# Autodesk Inventor assembly: L1 Gearbox Assembly
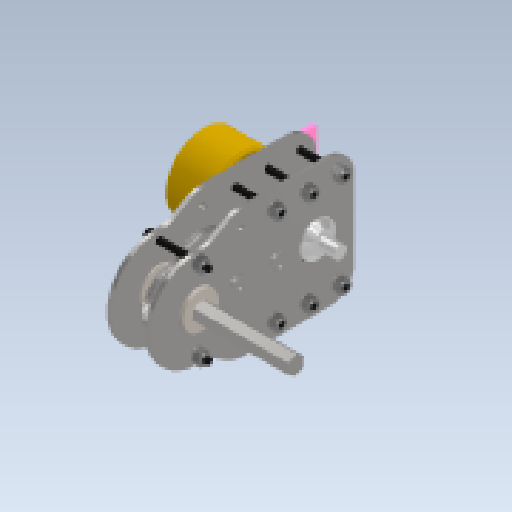
[picture p0: Inventor's stored thumbnail of the model, 512x512]
Saved by Autodesk Inventor 2023 (Build 270158000, 158)
## iProperties
Created: 2023-02-14
Part Number: L1 Gearbox Assembly
Document SubType Name: Assembly
Designer: Dave
Mass: 913.46 g
Surface Area: 1660.69 cm^2
Volume: 243.163 cm^3
Density: 3.75658 g/cm^3
Author: Dave
## Documents named in this file (16)
- C:\Users\Dave\Documents\GitHub\BehrendURCMechanical\CAD\Chassis V3\L1 Gearbox Assembly.iam
- C:\Users\Dave\Documents\GitHub\BehrendURCMechanical\CAD\Chassis\GearBox\Final Gears and Assemblies\CH-1-01-20T_Drive Gear.ipt
- C:\Users\Dave\Documents\GitHub\BehrendURCMechanical\CAD\Chassis\GearBox\Final Gears and Assemblies\CH-1-01-60T_Output.ipt
- C:\Users\Dave\Documents\GitHub\BehrendURCMechanical\CAD\Chassis\GearBox\Final Gears and Assemblies\CH-1-01-20T_Idler.ipt
- C:\Users\Dave\Documents\GitHub\BehrendURCMechanical\CAD\Chassis\GearBox\Final Gears and Assemblies\CH-1-01-60T_Idler.ipt
- C:\Users\Dave\Documents\GitHub\BehrendURCMechanical\CAD\Chassis\GearBox\Housing\CH-1-02-RearGearboxHousingMotorSide.ipt
- C:\Users\Dave\Documents\GitHub\BehrendURCMechanical\CAD\Chassis\GearBox\Drive Motor Shaft Coupler.ipt
- C:\Users\Dave\Documents\GitHub\BehrendURCMechanical\CAD\Chassis\GearBox\Ch-1-01-0.5x4.5HexShaft.ipt
- C:\Users\Dave\Documents\GitHub\BehrendURCMechanical\CAD\Chassis\GearBox\CH-1-01-0.25x1.875SmoothShaft.ipt
- C:\Users\Dave\Documents\GitHub\BehrendURCMechanical\CAD\Chassis\GearBox\CH-1-01-0.5HexBearing.ipt
- C:\Users\Dave\Documents\GitHub\BehrendURCMechanical\CAD\Chassis\GearBox\CH-1-01-0.25IDSmoothBoreBearing.ipt
- C:\Users\Dave\Documents\GitHub\BehrendURCMechanical\CAD\Chassis V3\DriveMotorAssem\DriveMotorAssem.iam
- C:\Users\Dave\Downloads\91251A252_Black-Oxide Alloy Steel Socket Head Screw.ipt
- C:\Users\Dave\Downloads\91831A011_18-8 Stainless Steel Nylon-Insert Locknut (1).ipt
- C:\Users\Dave\Documents\GitHub\BehrendURCMechanical\CAD\Chassis V3\90107A011_316 Stainless Steel Washer.ipt
- C:\Users\Dave\Documents\GitHub\BehrendURCMechanical\CAD\Chassis V3\L1Plate.ipt
## Components (53 placed, 15 different names)
1. CH-1-01-20T_Drive Gear:1 — Insert:16
2. CH-1-01-60T_Output:1 — Mate:17, Flush:6
3. CH-1-01-20T_Idler:1 — Mate:21, Flush:5
4. CH-1-01-60T_Idler:1 — Mate:18, Mate:19, Mate:20, Flush:5
5. CH-1-01-20T_Idler:2 — Mate:19, Mate:22, Flush:6
6. CH-1-01-60T_Idler:2 — Mate:10, Mate:11
7. CH-1-02-RearGearboxHousingMotorSide:1 — Angle:1, Flush:1, Flush:2, Insert:6, Insert:7, Insert:10, Mate:26, Insert:35, Insert:36, Insert:37, Insert:40, Insert:41, Insert:42, Flush:9
8. CH-1-02-RearGearboxHousingMotorSide:2 — Flush:1, Flush:2, Insert:8, Insert:9, Insert:11, Flush:10
9. Drive Motor Shaft Coupler:1 — Insert:16, Mate:26, Mate:27, Mate:31
10. DriveMotorAssem:1 [sub-assembly] — Mate:27, Insert:59, Insert:60, Insert:61, Insert:62, Insert:63, Insert:64, Insert:65
11. Ch-1-01-0.5x4.5HexShaft:1 — Mate:8, Mate:9, Flush:8
12. CH-1-01-0.25x1.875SmoothShaft:1 — Insert:13
13. CH-1-01-0.25x1.875SmoothShaft:2 — Insert:12, Flush:4
14. CH-1-01-0.5HexBearing:1 — Insert:11, Mate:17, Flush:8
15. CH-1-01-0.5HexBearing:2 — Insert:10, Mate:8, Mate:9, Mate:29, Mate:30
16. CH-1-01-0.25IDSmoothBoreBearing:1 — Insert:6, Insert:12
17. CH-1-01-0.25IDSmoothBoreBearing:2 — Insert:7, Insert:13, Mate:11
18. CH-1-01-0.25IDSmoothBoreBearing:3 — Insert:8, Flush:4, Mate:18, Mate:20, Mate:22
19. CH-1-01-0.25IDSmoothBoreBearing:4 — Insert:9, Mate:10, Mate:21
20. 91251A252_Black-Oxide Alloy Steel Socket Head Screw:1 — Insert:23, Mate:28
21. 91831A011_18-8 Stainless Steel Nylon-Insert Locknut (1):1 — Insert:54
22. 91251A252_Black-Oxide Alloy Steel Socket Head Screw:2 — Insert:24
23. 91831A011_18-8 Stainless Steel Nylon-Insert Locknut (1):2 — Insert:48
24. 91251A252_Black-Oxide Alloy Steel Socket Head Screw:3 — Insert:25
25. 91831A011_18-8 Stainless Steel Nylon-Insert Locknut (1):3 — Insert:49
26. 91251A252_Black-Oxide Alloy Steel Socket Head Screw:4 — Insert:52
27. 91831A011_18-8 Stainless Steel Nylon-Insert Locknut (1):4 — Insert:50
28. 91251A252_Black-Oxide Alloy Steel Socket Head Screw:5 — Insert:31
29. 91831A011_18-8 Stainless Steel Nylon-Insert Locknut (1):5 — Insert:43
30. 91251A252_Black-Oxide Alloy Steel Socket Head Screw:6 — Insert:32
31. 91831A011_18-8 Stainless Steel Nylon-Insert Locknut (1):6 — Insert:44
32. 91251A252_Black-Oxide Alloy Steel Socket Head Screw:7 — Insert:33
33. 91831A011_18-8 Stainless Steel Nylon-Insert Locknut (1):7 — Insert:45
34. 91251A252_Black-Oxide Alloy Steel Socket Head Screw:8 — Insert:56
35. 91831A011_18-8 Stainless Steel Nylon-Insert Locknut (1):8 — Insert:58
36. 90107A011_316 Stainless Steel Washer:1 — Insert:23, Insert:61
37. 90107A011_316 Stainless Steel Washer:2 — Insert:42, Insert:50
38. 90107A011_316 Stainless Steel Washer:3 — Insert:41, Insert:49
39. 90107A011_316 Stainless Steel Washer:4 — Insert:24, Insert:60
40. 90107A011_316 Stainless Steel Washer:5 — Insert:40, Insert:48
41. 90107A011_316 Stainless Steel Washer:6 — Insert:25, Insert:59
42. 90107A011_316 Stainless Steel Washer:7 — Insert:53, Insert:54
43. 90107A011_316 Stainless Steel Washer:8 — Insert:51, Insert:52
44. 90107A011_316 Stainless Steel Washer:9 — Insert:57, Insert:58
45. 90107A011_316 Stainless Steel Washer:10 — Insert:55, Insert:56
46. 90107A011_316 Stainless Steel Washer:11 — Insert:37, Insert:45
47. 90107A011_316 Stainless Steel Washer:12 — Insert:33, Insert:65
48. 90107A011_316 Stainless Steel Washer:13 — Insert:36, Insert:44
49. 90107A011_316 Stainless Steel Washer:14 — Insert:32, Insert:64
50. 90107A011_316 Stainless Steel Washer:15 — Insert:35, Insert:43
51. 90107A011_316 Stainless Steel Washer:16 — Insert:31, Insert:63
52. L1Plate:1 — Mate:28, Flush:9, Mate:29, Insert:53, Insert:57
53. L1Plate:2 — Mate:30, Mate:31, Flush:10, Insert:51, Insert:55, Insert:62
## Relationships (67: Insert 42, Mate 16, Flush 8, Angle 1)
- Angle:1 (0 deg): CH-1-02-RearGearboxHousingMotorSide:1
- Flush:1: CH-1-02-RearGearboxHousingMotorSide:1 ↔ CH-1-02-RearGearboxHousingMotorSide:2
- Flush:2: CH-1-02-RearGearboxHousingMotorSide:1 ↔ CH-1-02-RearGearboxHousingMotorSide:2
- Insert:6: CH-1-02-RearGearboxHousingMotorSide:1 ↔ CH-1-01-0.25IDSmoothBoreBearing:1
- Insert:7: CH-1-02-RearGearboxHousingMotorSide:1 ↔ CH-1-01-0.25IDSmoothBoreBearing:2
- Insert:8: CH-1-02-RearGearboxHousingMotorSide:2 ↔ CH-1-01-0.25IDSmoothBoreBearing:3
- Insert:9: CH-1-02-RearGearboxHousingMotorSide:2 ↔ CH-1-01-0.25IDSmoothBoreBearing:4
- Insert:10: CH-1-02-RearGearboxHousingMotorSide:1 ↔ CH-1-01-0.5HexBearing:2
- Insert:11: CH-1-02-RearGearboxHousingMotorSide:2 ↔ CH-1-01-0.5HexBearing:1
- Mate:8: Ch-1-01-0.5x4.5HexShaft:1 ↔ CH-1-01-0.5HexBearing:2
- Mate:9: Ch-1-01-0.5x4.5HexShaft:1 ↔ CH-1-01-0.5HexBearing:2
- Insert:12: CH-1-01-0.25x1.875SmoothShaft:2 ↔ CH-1-01-0.25IDSmoothBoreBearing:1
- Insert:13: CH-1-01-0.25x1.875SmoothShaft:1 ↔ CH-1-01-0.25IDSmoothBoreBearing:2
- Mate:10: CH-1-01-60T_Idler:2 ↔ CH-1-01-0.25IDSmoothBoreBearing:4
- Mate:11: CH-1-01-60T_Idler:2 ↔ CH-1-01-0.25IDSmoothBoreBearing:2
- Flush:4: CH-1-01-0.25x1.875SmoothShaft:2 ↔ CH-1-01-0.25IDSmoothBoreBearing:3
- Mate:17: CH-1-01-60T_Output:1 ↔ CH-1-01-0.5HexBearing:1
- Mate:18: CH-1-01-60T_Idler:1 ↔ CH-1-01-0.25IDSmoothBoreBearing:3
- Mate:19: CH-1-01-60T_Idler:1 ↔ CH-1-01-20T_Idler:2
- Mate:20: CH-1-01-60T_Idler:1 ↔ CH-1-01-0.25IDSmoothBoreBearing:3
- Mate:21: CH-1-01-20T_Idler:1 ↔ CH-1-01-0.25IDSmoothBoreBearing:4
- Flush:5: CH-1-01-20T_Idler:1 ↔ CH-1-01-60T_Idler:1
- Mate:22: CH-1-01-20T_Idler:2 ↔ CH-1-01-0.25IDSmoothBoreBearing:3
- Flush:6: CH-1-01-60T_Output:1 ↔ CH-1-01-20T_Idler:2
- Flush:8: Ch-1-01-0.5x4.5HexShaft:1 ↔ CH-1-01-0.5HexBearing:1
- Insert:16: CH-1-01-20T_Drive Gear:1 ↔ Drive Motor Shaft Coupler:1
- Mate:26: CH-1-02-RearGearboxHousingMotorSide:1 ↔ Drive Motor Shaft Coupler:1
- Mate:27: Drive Motor Shaft Coupler:1 ↔ DriveMotorAssem:1
- Insert:23: 91251A252_Black-Oxide Alloy Steel Socket Head Screw:1 ↔ 90107A011_316 Stainless Steel Washer:1
- Insert:24: 91251A252_Black-Oxide Alloy Steel Socket Head Screw:2 ↔ 90107A011_316 Stainless Steel Washer:4
- Insert:25: 91251A252_Black-Oxide Alloy Steel Socket Head Screw:3 ↔ 90107A011_316 Stainless Steel Washer:6
- Insert:31: 91251A252_Black-Oxide Alloy Steel Socket Head Screw:5 ↔ 90107A011_316 Stainless Steel Washer:16
- Insert:32: 91251A252_Black-Oxide Alloy Steel Socket Head Screw:6 ↔ 90107A011_316 Stainless Steel Washer:14
- Insert:33: 91251A252_Black-Oxide Alloy Steel Socket Head Screw:7 ↔ 90107A011_316 Stainless Steel Washer:12
- Insert:35: CH-1-02-RearGearboxHousingMotorSide:1 ↔ 90107A011_316 Stainless Steel Washer:15
- Insert:36: CH-1-02-RearGearboxHousingMotorSide:1 ↔ 90107A011_316 Stainless Steel Washer:13
- Insert:37: CH-1-02-RearGearboxHousingMotorSide:1 ↔ 90107A011_316 Stainless Steel Washer:11
- Insert:40: CH-1-02-RearGearboxHousingMotorSide:1 ↔ 90107A011_316 Stainless Steel Washer:5
- Insert:41: CH-1-02-RearGearboxHousingMotorSide:1 ↔ 90107A011_316 Stainless Steel Washer:3
- Insert:42: CH-1-02-RearGearboxHousingMotorSide:1 ↔ 90107A011_316 Stainless Steel Washer:2
- Insert:43: 91831A011_18-8 Stainless Steel Nylon-Insert Locknut (1):5 ↔ 90107A011_316 Stainless Steel Washer:15
- Insert:44: 91831A011_18-8 Stainless Steel Nylon-Insert Locknut (1):6 ↔ 90107A011_316 Stainless Steel Washer:13
- Insert:45: 91831A011_18-8 Stainless Steel Nylon-Insert Locknut (1):7 ↔ 90107A011_316 Stainless Steel Washer:11
- Insert:48: 91831A011_18-8 Stainless Steel Nylon-Insert Locknut (1):2 ↔ 90107A011_316 Stainless Steel Washer:5
- Insert:49: 91831A011_18-8 Stainless Steel Nylon-Insert Locknut (1):3 ↔ 90107A011_316 Stainless Steel Washer:3
- Insert:50: 91831A011_18-8 Stainless Steel Nylon-Insert Locknut (1):4 ↔ 90107A011_316 Stainless Steel Washer:2
- Mate:28: 91251A252_Black-Oxide Alloy Steel Socket Head Screw:1 ↔ L1Plate:1
- Flush:9: CH-1-02-RearGearboxHousingMotorSide:1 ↔ L1Plate:1
- Mate:29: CH-1-01-0.5HexBearing:2 ↔ L1Plate:1
- Mate:30: CH-1-01-0.5HexBearing:2 ↔ L1Plate:2
- Mate:31: Drive Motor Shaft Coupler:1 ↔ L1Plate:2
- Flush:10: CH-1-02-RearGearboxHousingMotorSide:2 ↔ L1Plate:2
- Insert:51: 90107A011_316 Stainless Steel Washer:8 ↔ L1Plate:2
- Insert:52: 91251A252_Black-Oxide Alloy Steel Socket Head Screw:4 ↔ 90107A011_316 Stainless Steel Washer:8
- Insert:53: 90107A011_316 Stainless Steel Washer:7 ↔ L1Plate:1
- Insert:54: 91831A011_18-8 Stainless Steel Nylon-Insert Locknut (1):1 ↔ 90107A011_316 Stainless Steel Washer:7
- Insert:55: 90107A011_316 Stainless Steel Washer:10 ↔ L1Plate:2
- Insert:56: 91251A252_Black-Oxide Alloy Steel Socket Head Screw:8 ↔ 90107A011_316 Stainless Steel Washer:10
- Insert:57: 90107A011_316 Stainless Steel Washer:9 ↔ L1Plate:1
- Insert:58: 91831A011_18-8 Stainless Steel Nylon-Insert Locknut (1):8 ↔ 90107A011_316 Stainless Steel Washer:9
- Insert:59: DriveMotorAssem:1 ↔ 90107A011_316 Stainless Steel Washer:6
- Insert:60: DriveMotorAssem:1 ↔ 90107A011_316 Stainless Steel Washer:4
- Insert:61: DriveMotorAssem:1 ↔ 90107A011_316 Stainless Steel Washer:1
- Insert:62: DriveMotorAssem:1 ↔ L1Plate:2
- Insert:63: DriveMotorAssem:1 ↔ 90107A011_316 Stainless Steel Washer:16
- Insert:64: DriveMotorAssem:1 ↔ 90107A011_316 Stainless Steel Washer:14
- Insert:65: DriveMotorAssem:1 ↔ 90107A011_316 Stainless Steel Washer:12
